# Autodesk Inventor assembly: 組合1
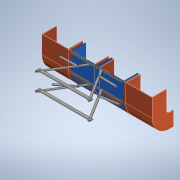
[picture p0: Inventor's stored thumbnail of the model, 180x180]
Saved by Autodesk Inventor 2022.3 (Build 263350000, 350)
## iProperties
Created: 2023-04-16
Part Number: 組合1
Document SubType Name: Assembly
Designer: JOU
Author: JOU
## Documents named in this file (6)
- D:\Areo_Rider_Cabin\test\組合1.iam
- D:\Areo_Rider_Cabin\test\零件1.ipt
- D:\Areo_Rider_Cabin\test\零件2.ipt
- D:\Areo_Rider_Cabin\test\零件3.ipt
- D:\Areo_Rider_Cabin\test\零件4.ipt
- D:\Areo_Rider_Cabin\Airfoil & Nuzzle\nuzzle\nuzzle_v2_0327.ipt
## Components (15 placed, 5 different names)
1. 零件1:1 — 插入:2, 插入:5, 齊平:6, 齊平:7
2. 零件2:1 — 插入:5, 插入:6, 相切:1
3. 零件2:2 — 插入:2, 插入:4, 相切:2, 貼合:13
4. 零件3:1 — 貼合:9, 插入:6
5. 零件3:2 — 插入:4, 貼合:8
6. 零件4:1 — 貼合:10, 貼合:11, 貼合:12, 相切:1, 相切:2, 貼合:13
7. nuzzle_v2_0327:1 — 貼合:7, 齊平:2, 齊平:3, 齊平:4, 齊平:5, 貼合:10, 貼合:11, 貼合:12, 貼合:15, 貼合:16, 貼合:17
8. nuzzle_v2_0327:2 — 齊平:3, 齊平:4, 貼合:8
9. nuzzle_v2_0327:3 — 齊平:2, 齊平:5, 貼合:9
10. 零件1:2 — 齊平:6, 齊平:7
11. 零件2:3
12. 零件2:4
13. 零件3:3
14. 零件3:4
15. 零件4:2 — 貼合:15, 貼合:16, 貼合:17
## Relationships (29: Mate 11, Insert 8, Flush 6, Tangent 4)
- 插入:2 [Insert]: 零件1:1 ↔ 零件2:2
- 插入:4 [Insert]: 零件2:2 ↔ 零件3:2
- 貼合:7 [Mate] (5 mm): nuzzle_v2_0327:1
- 齊平:2 [Flush]: nuzzle_v2_0327:1 ↔ nuzzle_v2_0327:3
- 齊平:3 [Flush]: nuzzle_v2_0327:1 ↔ nuzzle_v2_0327:2
- 齊平:4 [Flush]: nuzzle_v2_0327:1 ↔ nuzzle_v2_0327:2
- 齊平:5 [Flush]: nuzzle_v2_0327:1 ↔ nuzzle_v2_0327:3
- 貼合:8 [Mate]: 零件3:2 ↔ nuzzle_v2_0327:2
- 貼合:9 [Mate]: 零件3:1 ↔ nuzzle_v2_0327:3
- 貼合:10 [Mate]: 零件4:1 ↔ nuzzle_v2_0327:1
- 貼合:11 [Mate]: 零件4:1 ↔ nuzzle_v2_0327:1
- 貼合:12 [Mate]: 零件4:1 ↔ nuzzle_v2_0327:1
- 插入:5 [Insert]: 零件1:1 ↔ 零件2:1
- 插入:6 [Insert]: 零件2:1 ↔ 零件3:1
- 相切:1 [Tangent]: 零件2:1 ↔ 零件4:1
- 相切:2 [Tangent]: 零件2:2 ↔ 零件4:1
- 貼合:13 [Mate]: 零件2:2 ↔ 零件4:1
- [Insert]: 零件1:2 ↔ 零件2:4
- [Insert]: 零件2:4 ↔ 零件3:4
- [Insert]: 零件1:2 ↔ 零件2:3
- [Insert]: 零件2:3 ↔ 零件3:3
- [Tangent]: 零件2:3 ↔ 零件4:2
- [Tangent]: 零件2:4 ↔ 零件4:2
- [Mate]: 零件2:4 ↔ 零件4:2
- 貼合:15 [Mate]: nuzzle_v2_0327:1 ↔ 零件4:2
- 貼合:16 [Mate]: nuzzle_v2_0327:1 ↔ 零件4:2
- 貼合:17 [Mate]: nuzzle_v2_0327:1 ↔ 零件4:2
- 齊平:6 [Flush]: 零件1:1 ↔ 零件1:2
- 齊平:7 [Flush]: 零件1:1 ↔ 零件1:2
## Named parameters: d28_d1 = 0 mm, d29_d3 = 0 mm, d30_d23 = 0 mm, d31_d24 = 0 mm, d32_d25 = 0 mm, d33_d26 = 0 mm, d34_d27 = 0 mm
